# Autodesk Inventor assembly: Cube 1x1 V5 (Objective)
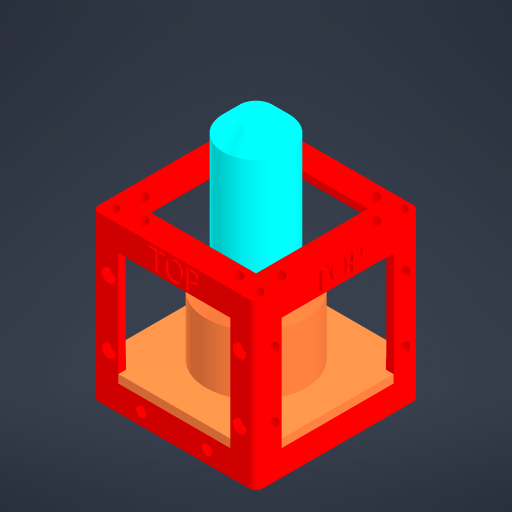
[picture p0: Inventor's stored thumbnail of the model, 512x512]
Saved by Autodesk Inventor 2023.4 (Build 274418000, 418)
## iProperties
Created: 2022-08-13
Part Number: Cube 1x1 V5 (Objective)
Document SubType Name: Assembly
Designer: xSibe
Author: xSibe
## Documents named in this file (4)
- C:\.Laptop\.Work\Projects\Project Protocube\Protocube\CAD, STL, OBJ Files\1 CAD\Objective\Cube 1x1 V5 (Objective).iam
- C:\.Laptop\.Work\Projects\Project Protocube\Protocube\CAD, STL, OBJ Files\1 CAD\Objective\Objective Mount.ipt
- C:\.Laptop\.Work\Projects\Project Protocube\Protocube\CAD, STL, OBJ Files\1 CAD\Objective\Objective.ipt
- C:\.Laptop\.Work\Projects\Project Protocube\Protocube\CAD, STL, OBJ Files\1 CAD\Cubes\Cube 1x1 V5.iam
## Components (3 placed, 3 different names)
1. Objective Mount:1 — Mate:4, Mate:5
2. Objective:1 — Mate:4, Mate:5, Mate:6
3. Cube 1x1 V5:1 [sub-assembly]
## Relationships (3: Mate 3)
- Mate:4: Objective Mount:1 ↔ Objective:1
- Mate:5: Objective Mount:1 ↔ Objective:1
- Mate:6: Objective:1
